# Autodesk Inventor assembly: long covering
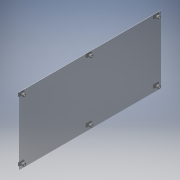
[picture p0: Inventor's stored thumbnail of the model, 180x180]
Saved by Autodesk Inventor 2016 (Build 200138000, 138)
## iProperties
Created: 2016-08-02
Part Number: long covering
Document SubType Name: Assembly
Designer: Jonathan
Author: Jonathan
## Documents named in this file (4)
- C:\Users\Jonathan\Desktop\Models\Three Panel Detector\frame\separator\long covering.iam
- C:\Users\Jonathan\Desktop\Models\Three Panel Detector\frame\separator\long covering.ipt
- C:\Users\Jonathan\Desktop\Models\Three Panel Detector\frame\brackets\m5x6.ipt
- C:\Users\Jonathan\Desktop\Models\Three Panel Detector\frame\brackets\m5TNut.ipt
## Components (13 placed, 3 different names)
1. long covering:1 — Mate:1, Mate:2, Angle:1, Mate:4, Angle:2
2. m5x6:1 — Mate:1, Mate:2, Mate:3, Angle:2
3. m5TNut:1 — Mate:3, Angle:1, Mate:4
4. m5x6:2
5. m5TNut:2
6. m5x6:3
7. m5TNut:3
8. m5x6:4
9. m5TNut:4
10. m5x6:5
11. m5TNut:5
12. m5x6:6
13. m5TNut:6
## Component patterns: (6 elements, first: m5x6:1 + m5TNut:1)
## Relationships (6: Mate 4, Angle 2)
- Mate:1: long covering:1 ↔ m5x6:1
- Mate:2: long covering:1 ↔ m5x6:1
- Mate:3: m5x6:1 ↔ m5TNut:1
- Angle:1 (0 deg): long covering:1 ↔ m5TNut:1
- Mate:4 (2 mm): long covering:1 ↔ m5TNut:1
- Angle:2 (0 deg): long covering:1 ↔ m5x6:1
